# Autodesk Inventor assembly: 000 Ensamblaje hw_DAA - BASIC - Cubo
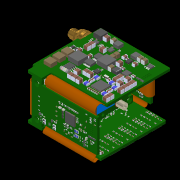
[picture p0: Inventor's stored thumbnail of the model, 180x180]
Saved by Autodesk Inventor 2018 (Build 220112000, 112)
## iProperties
Created: 2024-03-14
Part Number: 000 Ensamblaje hw_DAA - BASIC - Cubo
Document SubType Name: Assembly
Designer: cda1
Mass: 217.675 g
Surface Area: 967.459 cm^2
Volume: 79.0664 cm^3
Density: 2.75306 g/cm^3
Author: cda1
## Documents named in this file (12)
- C:\Users\cda1\Git\DAA\items\hw_DAA\variants\BASIC\3d\000 Ensamblaje hw_DAA - BASIC - Cubo.iam
- C:\Users\cda1\Git\DAA\items\hw_DAA\variants\BASIC\3d\000 Ensamblaje hw_DAA - PCB FPGA.iam
- C:\Users\cda1\Git\DAA\items\hw_DAA\variants\BASIC\3d\000 Ensamblaje hw_DAA - PCB Peripherals.iam
- C:\Users\cda1\Git\DAA\items\hw_DAA\variants\BASIC\3d\000 Ensamblaje hw_DAA - PCB MicroSD.iam
- C:\Users\cda1\Git\DAA\items\hw_DAA\variants\BASIC\3d\000 Ensamblaje hw_DAA - PCB Lemo.iam
- C:\Users\cda1\Git\DAA\items\hw_DAA\variants\BASIC\3d\000 Ensamblaje hw_DAA - PCB Sensor.iam
- C:\Users\cda1\Git\DAA\items\hw_DAA\variants\BASIC\3d\000 Ensamblaje hw_DAA - PCB Power.iam
- C:\Users\cda1\Git\DAA\items\3d_DAA\3d\3d_DAA - Flex 1.ipt
- C:\Users\cda1\Git\DAA\items\3d_DAA\3d\3d_DAA - Flex 2.ipt
- C:\Users\cda1\Git\DAA\items\3d_DAA\3d\3d_DAA - Flex 3.ipt
- C:\Users\cda1\Git\DAA\items\3d_DAA\3d\3d_DAA - Flex 4.ipt
- C:\Users\cda1\Git\DAA\items\3d_DAA\3d\3d_DAA - Flex 5.ipt
## Components (11 placed, 11 different names)
1. 000 Ensamblaje hw_DAA - PCB FPGA:1 [sub-assembly] — Ángulo:1, Ángulo:2, Ángulo:3, Ángulo:4, Ángulo:6, Coincidencia:161, Nivelación:57, Ángulo:22, Coincidencia:252, Coincidencia:255, Coincidencia:256, Coincidencia:257, Coincidencia:266, Coincidencia:267, Coincidencia:269, Coincidencia:270
2. 000 Ensamblaje hw_DAA - PCB Peripherals:1 [sub-assembly] — Ángulo:1, Coincidencia:33, Coincidencia:43, Coincidencia:246, Coincidencia:254, Coincidencia:256, Nivelación:65, Coincidencia:271
3. 000 Ensamblaje hw_DAA - PCB MicroSD:1 [sub-assembly] — Ángulo:2, Coincidencia:118, Nivelación:61, Ángulo:23, Nivelación:63, Coincidencia:255, Coincidencia:257, Coincidencia:268
4. 000 Ensamblaje hw_DAA - PCB Lemo:1 [sub-assembly] — Ángulo:3, Ángulo:4, Coincidencia:21, Nivelación:57, Nivelación:61, Nivelación:64, Coincidencia:252, Coincidencia:253, Coincidencia:258
5. 000 Ensamblaje hw_DAA - PCB Sensor:1 [sub-assembly] — Ángulo:6, Coincidencia:161, Ángulo:22, Nivelación:62, Coincidencia:245
6. 000 Ensamblaje hw_DAA - PCB Power:1 [sub-assembly] — Coincidencia:21, Nivelación:62, Coincidencia:253, Coincidencia:254, Nivelación:65, Coincidencia:312
7. 3d_DAA - Flex 1:1 — Nivelación:64, Coincidencia:246, Coincidencia:258
8. 3d_DAA - Flex 2:1 — Coincidencia:33, Coincidencia:43, Coincidencia:312
9. 3d_DAA - Flex 3:1 — Coincidencia:118, Ángulo:23, Nivelación:63, Coincidencia:245
10. 3d_DAA - Flex 4:1 — Coincidencia:266, Coincidencia:267, Coincidencia:268
11. 3d_DAA - Flex 5:1 — Coincidencia:269, Coincidencia:270, Coincidencia:271
## Relationships (34: Mate 21, Angle 7, Flush 6)
- Ángulo:1 [Angle] (90 deg): 000 Ensamblaje hw_DAA - PCB FPGA:1 ↔ 000 Ensamblaje hw_DAA - PCB Peripherals:1
- Ángulo:2 [Angle] (90 deg): 000 Ensamblaje hw_DAA - PCB FPGA:1 ↔ 000 Ensamblaje hw_DAA - PCB MicroSD:1
- Ángulo:3 [Angle] (90 deg): 000 Ensamblaje hw_DAA - PCB FPGA:1 ↔ 000 Ensamblaje hw_DAA - PCB Lemo:1
- Ángulo:4 [Angle] (0 deg): 000 Ensamblaje hw_DAA - PCB FPGA:1 ↔ 000 Ensamblaje hw_DAA - PCB Lemo:1
- Ángulo:6 [Angle] (90 deg): 000 Ensamblaje hw_DAA - PCB FPGA:1 ↔ 000 Ensamblaje hw_DAA - PCB Sensor:1
- Coincidencia:21 [Mate]: 000 Ensamblaje hw_DAA - PCB Lemo:1 ↔ 000 Ensamblaje hw_DAA - PCB Power:1
- Coincidencia:33 [Mate]: 000 Ensamblaje hw_DAA - PCB Peripherals:1 ↔ 3d_DAA - Flex 2:1
- Coincidencia:43 [Mate] (2.5 mm): 000 Ensamblaje hw_DAA - PCB Peripherals:1 ↔ 3d_DAA - Flex 2:1
- Coincidencia:118 [Mate]: 000 Ensamblaje hw_DAA - PCB MicroSD:1 ↔ 3d_DAA - Flex 3:1
- Coincidencia:161 [Mate]: 000 Ensamblaje hw_DAA - PCB FPGA:1 ↔ 000 Ensamblaje hw_DAA - PCB Sensor:1
- Nivelación:57 [Flush]: 000 Ensamblaje hw_DAA - PCB FPGA:1 ↔ 000 Ensamblaje hw_DAA - PCB Lemo:1
- Nivelación:61 [Flush]: 000 Ensamblaje hw_DAA - PCB MicroSD:1 ↔ 000 Ensamblaje hw_DAA - PCB Lemo:1
- Ángulo:22 [Angle] (0 deg): 000 Ensamblaje hw_DAA - PCB FPGA:1 ↔ 000 Ensamblaje hw_DAA - PCB Sensor:1
- Ángulo:23 [Angle] (0 deg): 000 Ensamblaje hw_DAA - PCB MicroSD:1 ↔ 3d_DAA - Flex 3:1
- Nivelación:62 [Flush] (-23 mm): 000 Ensamblaje hw_DAA - PCB Sensor:1 ↔ 000 Ensamblaje hw_DAA - PCB Power:1
- Nivelación:63 [Flush] (8.2 mm): 000 Ensamblaje hw_DAA - PCB MicroSD:1 ↔ 3d_DAA - Flex 3:1
- Coincidencia:245 [Mate]: 000 Ensamblaje hw_DAA - PCB Sensor:1 ↔ 3d_DAA - Flex 3:1
- Nivelación:64 [Flush] (7.3 mm): 000 Ensamblaje hw_DAA - PCB Lemo:1 ↔ 3d_DAA - Flex 1:1
- Coincidencia:246 [Mate]: 000 Ensamblaje hw_DAA - PCB Peripherals:1 ↔ 3d_DAA - Flex 1:1
- Coincidencia:252 [Mate]: 000 Ensamblaje hw_DAA - PCB FPGA:1 ↔ 000 Ensamblaje hw_DAA - PCB Lemo:1
- Coincidencia:253 [Mate]: 000 Ensamblaje hw_DAA - PCB Lemo:1 ↔ 000 Ensamblaje hw_DAA - PCB Power:1
- Coincidencia:254 [Mate]: 000 Ensamblaje hw_DAA - PCB Peripherals:1 ↔ 000 Ensamblaje hw_DAA - PCB Power:1
- Coincidencia:255 [Mate]: 000 Ensamblaje hw_DAA - PCB FPGA:1 ↔ 000 Ensamblaje hw_DAA - PCB MicroSD:1
- Coincidencia:256 [Mate]: 000 Ensamblaje hw_DAA - PCB FPGA:1 ↔ 000 Ensamblaje hw_DAA - PCB Peripherals:1
- Coincidencia:257 [Mate]: 000 Ensamblaje hw_DAA - PCB FPGA:1 ↔ 000 Ensamblaje hw_DAA - PCB MicroSD:1
- Nivelación:65 [Flush]: 000 Ensamblaje hw_DAA - PCB Peripherals:1 ↔ 000 Ensamblaje hw_DAA - PCB Power:1
- Coincidencia:258 [Mate]: 000 Ensamblaje hw_DAA - PCB Lemo:1 ↔ 3d_DAA - Flex 1:1
- Coincidencia:266 [Mate]: 000 Ensamblaje hw_DAA - PCB FPGA:1 ↔ 3d_DAA - Flex 4:1
- Coincidencia:267 [Mate] (1.5 mm): 000 Ensamblaje hw_DAA - PCB FPGA:1 ↔ 3d_DAA - Flex 4:1
- Coincidencia:268 [Mate]: 000 Ensamblaje hw_DAA - PCB MicroSD:1 ↔ 3d_DAA - Flex 4:1
- Coincidencia:269 [Mate]: 000 Ensamblaje hw_DAA - PCB FPGA:1 ↔ 3d_DAA - Flex 5:1
- Coincidencia:270 [Mate] (2.5 mm): 000 Ensamblaje hw_DAA - PCB FPGA:1 ↔ 3d_DAA - Flex 5:1
- Coincidencia:271 [Mate]: 000 Ensamblaje hw_DAA - PCB Peripherals:1 ↔ 3d_DAA - Flex 5:1
- Coincidencia:312 [Mate]: 000 Ensamblaje hw_DAA - PCB Power:1 ↔ 3d_DAA - Flex 2:1
